# Autodesk Inventor assembly: base
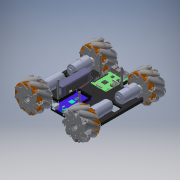
[picture p0: Inventor's stored thumbnail of the model, 180x180]
Saved by Autodesk Inventor 2017 (Build 210142000, 142)
## iProperties
Created: 2017-03-20
Part Number: base
Document SubType Name: Assembly
Designer: Naga
Author: Naga
## Documents named in this file (9)
- E:\GDrive\IEEE CS\SoutheastCon2017\Cad\base.iam
- E:\GDrive\IEEE CS\SoutheastCon2017\Cad\Chassis\BottomPlateV3.ipt
- E:\GDrive\IEEE CS\SoutheastCon2017\Cad\Electronics\RaspberryPi2 STEP214.iam
- E:\GDrive\IEEE CS\SoutheastCon2017\Cad\Electronics\Arduino Mega 2560.ipt
- E:\GDrive\IEEE CS\SoutheastCon2017\Cad\Electronics\kangarooSaberTooth.iam
- E:\GDrive\IEEE CS\SoutheastCon2017\Cad\Chassis\postSpacer.ipt
- E:\GDrive\IEEE CS\SoutheastCon2017\Cad\Motors\100mm Aluminum Mecanum wheels.iam
- E:\GDrive\IEEE CS\SoutheastCon2017\Cad\Motors\37DEncoderAlBlock.iam
- E:\GDrive\IEEE CS\SoutheastCon2017\Cad\Electronics\2200mAh LiPo.iam
## Components (18 placed, 8 different names)
1. BottomPlateV3:1 — Flush:1, Mate:1, Flush:2, Mate:2, Flush:3, Mate:3, Flush:4, Flush:5, Mate:4, Mate:7, Flush:6, Flush:7, Flush:8, Flush:9, Mate:8, Mate:9, Mate:10, Mate:11, Mate:12, Mate:13, Mate:14, Mate:15, Mate:20, Mate:21, Mate:22, Mate:23, Mate:24, Mate:25, Mate:26, Mate:27, Mate:28, Mate:37, Mate:38
2. RaspberryPi2 STEP214:1 [sub-assembly] — Flush:2, Mate:2, Flush:5
3. Arduino Mega 2560:1 — Flush:3, Mate:3, Flush:4
4. kangarooSaberTooth:1 [sub-assembly] — Mate:4, Flush:8, Flush:9
5. kangarooSaberTooth:2 [sub-assembly] — Mate:7, Flush:6, Flush:7
6. postSpacer:1 — Mate:11, Mate:15
7. postSpacer:2 — Mate:10, Mate:14
8. postSpacer:3 — Mate:12, Mate:13
9. postSpacer:4 — Mate:8, Mate:9
10. 100mm Aluminum Mecanum wheels:1 [sub-assembly] — Mate:29, Mate:35
11. 100mm Aluminum Mecanum wheels:2 [sub-assembly] — Mate:31, Mate:34
12. 100mm Aluminum Mecanum wheels:3 [sub-assembly] — Mate:30, Mate:36
13. 100mm Aluminum Mecanum wheels:4 [sub-assembly] — Mate:32, Mate:33
14. 37DEncoderAlBlock:1 [sub-assembly] — Mate:24, Mate:25, Flush:11, Mate:29, Mate:35
15. 37DEncoderAlBlock:2 [sub-assembly] — Mate:26, Mate:27, Flush:12, Mate:31, Mate:34
16. 37DEncoderAlBlock:3 [sub-assembly] — Mate:22, Mate:23, Flush:10, Mate:30, Mate:36
17. 37DEncoderAlBlock:4 [sub-assembly] — Mate:20, Mate:21, Flush:10, Flush:11, Flush:12, Mate:28, Mate:32, Mate:33
18. 2200mAh LiPo:1 [sub-assembly] — Mate:38
## Relationships (44: Mate 32, Flush 12)
- Flush:1: BottomPlateV3:1
- Mate:1: BottomPlateV3:1
- Flush:2: BottomPlateV3:1 ↔ RaspberryPi2 STEP214:1
- Mate:2: BottomPlateV3:1 ↔ RaspberryPi2 STEP214:1
- Flush:3: BottomPlateV3:1 ↔ Arduino Mega 2560:1
- Mate:3: BottomPlateV3:1 ↔ Arduino Mega 2560:1
- Flush:4 (1.8796 mm): BottomPlateV3:1 ↔ Arduino Mega 2560:1
- Flush:5 (0.5715 mm): BottomPlateV3:1 ↔ RaspberryPi2 STEP214:1
- Mate:4: BottomPlateV3:1 ↔ kangarooSaberTooth:1
- Mate:7: BottomPlateV3:1 ↔ kangarooSaberTooth:2
- Flush:6 (-47.752 mm): BottomPlateV3:1 ↔ kangarooSaberTooth:2
- Flush:7 (10.033 mm): BottomPlateV3:1 ↔ kangarooSaberTooth:2
- Flush:8 (47.752 mm): BottomPlateV3:1 ↔ kangarooSaberTooth:1
- Flush:9 (10.033 mm): BottomPlateV3:1 ↔ kangarooSaberTooth:1
- Mate:8: BottomPlateV3:1 ↔ postSpacer:4
- Mate:9: BottomPlateV3:1 ↔ postSpacer:4
- Mate:10: BottomPlateV3:1 ↔ postSpacer:2
- Mate:11: BottomPlateV3:1 ↔ postSpacer:1
- Mate:12: BottomPlateV3:1 ↔ postSpacer:3
- Mate:13: BottomPlateV3:1 ↔ postSpacer:3
- Mate:14: BottomPlateV3:1 ↔ postSpacer:2
- Mate:15: BottomPlateV3:1 ↔ postSpacer:1
- Mate:20: BottomPlateV3:1 ↔ 37DEncoderAlBlock:4
- Mate:21: BottomPlateV3:1 ↔ 37DEncoderAlBlock:4
- Mate:22: BottomPlateV3:1 ↔ 37DEncoderAlBlock:3
- Mate:23: BottomPlateV3:1 ↔ 37DEncoderAlBlock:3
- Mate:24: BottomPlateV3:1 ↔ 37DEncoderAlBlock:1
- Mate:25: BottomPlateV3:1 ↔ 37DEncoderAlBlock:1
- Mate:26: BottomPlateV3:1 ↔ 37DEncoderAlBlock:2
- Mate:27: BottomPlateV3:1 ↔ 37DEncoderAlBlock:2
- Flush:10: 37DEncoderAlBlock:3 ↔ 37DEncoderAlBlock:4
- Flush:11: 37DEncoderAlBlock:1 ↔ 37DEncoderAlBlock:4
- Flush:12: 37DEncoderAlBlock:2 ↔ 37DEncoderAlBlock:4
- Mate:28: BottomPlateV3:1 ↔ 37DEncoderAlBlock:4
- Mate:29: 100mm Aluminum Mecanum wheels:1 ↔ 37DEncoderAlBlock:1
- Mate:30: 100mm Aluminum Mecanum wheels:3 ↔ 37DEncoderAlBlock:3
- Mate:31: 100mm Aluminum Mecanum wheels:2 ↔ 37DEncoderAlBlock:2
- Mate:32: 100mm Aluminum Mecanum wheels:4 ↔ 37DEncoderAlBlock:4
- Mate:33: 100mm Aluminum Mecanum wheels:4 ↔ 37DEncoderAlBlock:4
- Mate:34: 100mm Aluminum Mecanum wheels:2 ↔ 37DEncoderAlBlock:2
- Mate:35: 100mm Aluminum Mecanum wheels:1 ↔ 37DEncoderAlBlock:1
- Mate:36: 100mm Aluminum Mecanum wheels:3 ↔ 37DEncoderAlBlock:3
- Mate:37 (31.75 mm): BottomPlateV3:1
- Mate:38: BottomPlateV3:1 ↔ 2200mAh LiPo:1
